# Autodesk Inventor assembly: photodetector_assembly
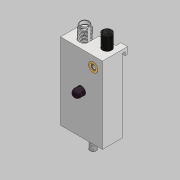
[picture p0: Inventor's stored thumbnail of the model, 180x180]
Saved by Autodesk Inventor 2021.4 (Build 254397000, 397)
## iProperties
Created: 2022-11-02
Part Number: photodetector_assembly
Document SubType Name: Assembly
Designer: Tilman Preuschoff
Author: Tilman Preuschoff
## Documents named in this file (10)
- C:\Users\Tilman Preuschoff\Documents\GitHub\SFH203_photodetector\case\assembly\photodetector_assembly.iam
- C:\Users\Tilman Preuschoff\Documents\GitHub\SFH203_photodetector\case\case.ipt
- C:\Users\Tilman Preuschoff\Documents\GitHub\SFH203_photodetector\case\assembly\SFH203_photodetector.iam
- C:\Users\Tilman Preuschoff\Documents\GitHub\SFH203_photodetector\case\assembly\cable.ipt
- C:\Users\Tilman Preuschoff\Documents\GitHub\SFH203_photodetector\case\assembly\ruthex_RX-M4Sx4.0_SHORT.iam
- C:\Users\Tilman Preuschoff\Documents\GitHub\SFH203_photodetector\case\cover.ipt
- C:\Users\Tilman Preuschoff\Documents\Inventor\Content Center Files\R2021\de-DE\DIN 125-2  A\DIN 125-2 - A 4,3A.ipt
- C:\Users\Tilman Preuschoff\Documents\Inventor\Content Center Files\R2021\de-DE\DIN 913\DIN 913 - M4 x 16.ipt
- C:\Users\Tilman Preuschoff\Documents\Inventor\Content Center Files\R2021\de-DE\DIN 913\DIN 913 - M4 x 6.ipt
- C:\Users\Tilman Preuschoff\Documents\GitHub\SFH203_photodetector\case\assembly\ruthex_RX-M2x4.iam
## Components (11 placed, 9 different names)
1. case:1 — Passend:1, Passend:3, Winkel:1, Winkel:5, Passend:15, Psend:16, Winkel:6, Drehbar:6, Zylindrisch:1, Zylindrisch:2, Passend:17, Fluchtend:1, Fluchtend:2, Drehbar:10, Drehbar:11
2. SFH203_photodetector:1 [sub-assembly] — Passend:15, Psend:16, Winkel:6
3. cable:1 — Winkel:5, Drehbar:6
4. ruthex_RX-M4Sx4.0_SHORT:1 [sub-assembly] — Zylindrisch:1, Drehbar:7
5. ruthex_RX-M4Sx4.0_SHORT:2 [sub-assembly] — Zylindrisch:2, Drehbar:9
6. cover:1 — Passend:17, Fluchtend:1, Fluchtend:2
7. DIN 125-2 A A 4,3:1 — Drehbar:7, Drehbar:8
8. DIN 913 M4 x 16:1 — Drehbar:8
9. DIN 913 M4 x 6:1 — Drehbar:9
10. ruthex_RX-M2x4:1 [sub-assembly] — Drehbar:10
11. ruthex_RX-M2x4:2 [sub-assembly] — Drehbar:11
## Relationships (18: RevoluteJoint 6, Mate 5, Angle 3, CylindricalJoint 2, Flush 2)
- Passend:1 [Mate]: case:1
- Passend:3 [Mate]: case:1
- Winkel:1 [Angle] (0 deg): case:1
- Winkel:5 [Angle] (0 deg): case:1 ↔ cable:1
- Passend:15 [Mate]: case:1 ↔ SFH203_photodetector:1
- Psend:16 [Mate]: case:1 ↔ SFH203_photodetector:1
- Winkel:6 [Angle] (0 deg): case:1 ↔ SFH203_photodetector:1
- Drehbar:6 [RevoluteJoint] (12 mm): case:1 ↔ cable:1
- Zylindrisch:1 [CylindricalJoint]: case:1 ↔ ruthex_RX-M4Sx4.0_SHORT:1
- Zylindrisch:2 [CylindricalJoint]: case:1 ↔ ruthex_RX-M4Sx4.0_SHORT:2
- Passend:17 [Mate]: case:1 ↔ cover:1
- Fluchtend:1 [Flush]: case:1 ↔ cover:1
- Fluchtend:2 [Flush]: case:1 ↔ cover:1
- Drehbar:7 [RevoluteJoint]: ruthex_RX-M4Sx4.0_SHORT:1 ↔ DIN 125-2 A A 4,3:1
- Drehbar:8 [RevoluteJoint] (7 mm): DIN 125-2 A A 4,3:1 ↔ DIN 913 M4 x 16:1
- Drehbar:9 [RevoluteJoint] (6 mm): ruthex_RX-M4Sx4.0_SHORT:2 ↔ DIN 913 M4 x 6:1
- Drehbar:10 [RevoluteJoint] (4 mm): case:1 ↔ ruthex_RX-M2x4:1
- Drehbar:11 [RevoluteJoint] (4 mm): case:1 ↔ ruthex_RX-M2x4:2
